# Autodesk Inventor assembly: BallBalancing_ASM01
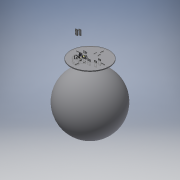
[picture p0: Inventor's stored thumbnail of the model, 180x180]
Saved by Autodesk Inventor 2016 (Build 200138000, 138)
## iProperties
Created: 2016-04-08
Part Number: BallBalancing_ASM01
Document SubType Name: Assembly
Designer: Admin
Author: Admin
## Documents named in this file (8)
- C:\Users\Admin\Documents\Inventor\BallBallerina\BallBalancing_ASM01.iam
- C:\Users\Admin\Documents\Inventor\BallBallerina\BallBallerina_BasePlate_v1.ipt
- C:\Users\Admin\Documents\Inventor\BallBallerina\BallBalancing_Hinge.ipt
- C:\Users\Admin\Documents\Inventor\BallBallerina\BallBalancing_MotorPlate.ipt
- C:\Users\Admin\Documents\Inventor\BallBallerina\BallBallancing_DCmotor.ipt
- C:\Users\Admin\Documents\Inventor\BallBallerina\BallBalancing_Wheel.ipt
- C:\Users\Admin\Documents\Inventor\BallBallerina\BallBallerina_Ball.ipt
- C:\Users\Admin\Documents\Inventor\BallBallerina\BallBallerina_LBracket.ipt
## Components (17 placed, 7 different names)
1. BallBallerina_BasePlate_v1:1 — Mate:1, Mate:2, Mate:3, Mate:4, Mate:5, Mate:6, Angle:1, Mate:7, Flush:2, Mate:17, Mate:18, Mate:19, Mate:20, Mate:21, Mate:22, Mate:23, Mate:24
2. BallBalancing_Hinge:1 — Mate:4, Mate:5, Flush:1, Flush:2, Mate:9, Mate:27, Mate:28, Mate:29, Mate:30
3. BallBalancing_Hinge:2 — Mate:6, Angle:1, Mate:7, Flush:1, Mate:8, Mate:25, Mate:26
4. BallBalancing_Hinge:3
5. BallBalancing_Hinge:4
6. BallBalancing_Hinge:5 — Mate:19, Mate:20
7. BallBalancing_Hinge:6 — Mate:17, Mate:18
8. BallBalancing_Hinge:7
9. BallBalancing_Hinge:8
10. BallBalancing_MotorPlate:1 — Mate:8, Mate:9, Mate:10, Mate:11, Mate:12
11. BallBallancing_DCmotor:1 — Mate:10, Mate:11, Mate:12, Mate:13, Mate:14
12. BallBalancing_Wheel:1 — Mate:13, Mate:14, Tangent:1, Tangent:2
13. BallBallerina_Ball:1 — Mate:15, Mate:16, Tangent:1, Tangent:2
14. BallBallerina_LBracket:1 — Mate:23, Mate:28, Mate:30
15. BallBallerina_LBracket:2 — Mate:22, Mate:27, Mate:29
16. BallBallerina_LBracket:3 — Mate:21, Mate:26
17. BallBallerina_LBracket:4 — Mate:24, Mate:25
## Relationships (35: Mate 30, Flush 2, Tangent 2, Angle 1)
- Mate:1: BallBallerina_BasePlate_v1:1
- Mate:2: BallBallerina_BasePlate_v1:1
- Mate:3: BallBallerina_BasePlate_v1:1
- Mate:4: BallBallerina_BasePlate_v1:1 ↔ BallBalancing_Hinge:1
- Mate:5: BallBallerina_BasePlate_v1:1 ↔ BallBalancing_Hinge:1
- Mate:6: BallBallerina_BasePlate_v1:1 ↔ BallBalancing_Hinge:2
- Angle:1 (0 deg): BallBallerina_BasePlate_v1:1 ↔ BallBalancing_Hinge:2
- Mate:7: BallBallerina_BasePlate_v1:1 ↔ BallBalancing_Hinge:2
- Flush:1: BallBalancing_Hinge:1 ↔ BallBalancing_Hinge:2
- Flush:2 (-13.5 mm): BallBallerina_BasePlate_v1:1 ↔ BallBalancing_Hinge:1
- Mate:8: BallBalancing_Hinge:2 ↔ BallBalancing_MotorPlate:1
- Mate:9: BallBalancing_Hinge:1 ↔ BallBalancing_MotorPlate:1
- Mate:10: BallBalancing_MotorPlate:1 ↔ BallBallancing_DCmotor:1
- Mate:11: BallBalancing_MotorPlate:1 ↔ BallBallancing_DCmotor:1
- Mate:12: BallBalancing_MotorPlate:1 ↔ BallBallancing_DCmotor:1
- Mate:13: BallBallancing_DCmotor:1 ↔ BallBalancing_Wheel:1
- Mate:14 (2 mm): BallBallancing_DCmotor:1 ↔ BallBalancing_Wheel:1
- Mate:15: BallBallerina_Ball:1
- Mate:16: BallBallerina_Ball:1
- Tangent:1: BallBalancing_Wheel:1 ↔ BallBallerina_Ball:1
- Tangent:2: BallBalancing_Wheel:1 ↔ BallBallerina_Ball:1
- Mate:17: BallBallerina_BasePlate_v1:1 ↔ BallBalancing_Hinge:6
- Mate:18: BallBallerina_BasePlate_v1:1 ↔ BallBalancing_Hinge:6
- Mate:19: BallBallerina_BasePlate_v1:1 ↔ BallBalancing_Hinge:5
- Mate:20: BallBallerina_BasePlate_v1:1 ↔ BallBalancing_Hinge:5
- Mate:21: BallBallerina_BasePlate_v1:1 ↔ BallBallerina_LBracket:3
- Mate:22: BallBallerina_BasePlate_v1:1 ↔ BallBallerina_LBracket:2
- Mate:23: BallBallerina_BasePlate_v1:1 ↔ BallBallerina_LBracket:1
- Mate:24: BallBallerina_BasePlate_v1:1 ↔ BallBallerina_LBracket:4
- Mate:25: BallBalancing_Hinge:2 ↔ BallBallerina_LBracket:4
- Mate:26: BallBalancing_Hinge:2 ↔ BallBallerina_LBracket:3
- Mate:27: BallBalancing_Hinge:1 ↔ BallBallerina_LBracket:2
- Mate:28: BallBalancing_Hinge:1 ↔ BallBallerina_LBracket:1
- Mate:29 (-0.5 mm): BallBalancing_Hinge:1 ↔ BallBallerina_LBracket:2
- Mate:30 (0.5 mm): BallBalancing_Hinge:1 ↔ BallBallerina_LBracket:1
